# Autodesk Inventor assembly: z_assembly
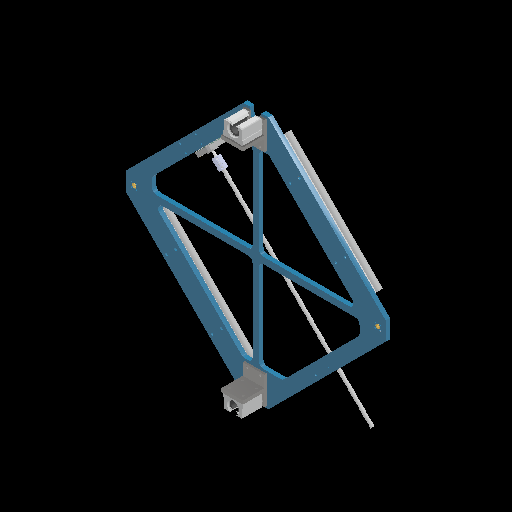
[picture p0: Inventor's stored thumbnail of the model, 512x512]
Saved by Autodesk Inventor 2026.1 (Build 301233000, 233)
## iProperties
Created: 2025-09-21
Part Number: z_assembly
Document SubType Name: Assembly
Designer: drago
Author: drago
## Documents named in this file (12)
- C:\Users\drago\Desktop\_QIST4500_Multidisciplinary_Team_Project\Proteox MX magnet positioner CAD\z_assembly\z_assembly.iam
- C:\Users\drago\Desktop\_QIST4500_Multidisciplinary_Team_Project\Proteox MX magnet positioner CAD\z_assembly\z_plate.ipt
- C:\Users\drago\Desktop\_QIST4500_Multidisciplinary_Team_Project\Proteox MX magnet positioner CAD\z_assembly\x_bearing_bracket.ipt
- C:\Users\drago\Desktop\_QIST4500_Multidisciplinary_Team_Project\Proteox MX magnet positioner CAD\z_assembly\z_bracket.ipt
- C:\Users\drago\Desktop\_QIST4500_Multidisciplinary_Team_Project\Proteox MX magnet positioner CAD\z_assembly\x_rail.ipt
- C:\Users\drago\Desktop\_QIST4500_Multidisciplinary_Team_Project\Proteox MX magnet positioner CAD\z_assembly\x_motor_bracket.ipt
- C:\Users\drago\Desktop\_QIST4500_Multidisciplinary_Team_Project\Proteox MX magnet positioner CAD\other_parts\KP08.iam
- C:\Users\drago\Desktop\_QIST4500_Multidisciplinary_Team_Project\Proteox MX magnet positioner CAD\other_parts\SBR16UU.ipt
- C:\Users\drago\Desktop\_QIST4500_Multidisciplinary_Team_Project\Proteox MX magnet positioner CAD\other_parts\Trapezoidal lead screw Nut tr8x8-4.ipt
- C:\Users\drago\Desktop\_QIST4500_Multidisciplinary_Team_Project\Proteox MX magnet positioner CAD\other_parts\Stepping_Motor_Nema17_34mm.ipt
- C:\Users\drago\Desktop\_QIST4500_Multidisciplinary_Team_Project\Proteox MX magnet positioner CAD\other_parts\5X8_COUPLER.ipt
- C:\Users\drago\Desktop\_QIST4500_Multidisciplinary_Team_Project\Proteox MX magnet positioner CAD\other_parts\Lead Screw 8mm-2.0 x 500mm.ipt
## Components (15 placed, 11 different names)
1. z_plate:1 — Mate:41, Mate:42, Mate:65, Mate:69, Mate:70, Mate:71, Mate:72, Mate:73, Mate:74, Mate:75, Mate:76, Mate:77, Mate:78, Mate:79, Mate:80, Mate:81, Mate:95, Mate:96, Mate:97, Mate:98, Mate:99, Mate:100, Mate:107, Mate:108, Mate:109
2. x_bearing_bracket:1 — Mate:65, Mate:84, Mate:85, Mate:86, Mate:109
3. z_bracket:1 — Mate:75, Mate:77, Mate:78, Mate:87, Mate:89, Mate:90
4. x_rail:1 — Mate:72, Mate:73, Mate:74
5. z_bracket:2 — Mate:76, Mate:79, Mate:80, Mate:88, Mate:91, Mate:92
6. x_rail:2 — Mate:69, Mate:70, Mate:71
7. x_motor_bracket:1 — Mate:81, Mate:101, Mate:102, Mate:103, Mate:107, Mate:108
8. KP08:1 [sub-assembly] — Mate:84, Mate:85, Mate:86, Mate:105
9. SBR16UU:1 — Mate:87, Mate:89, Mate:90
10. SBR16UU:2 — Mate:88, Mate:91, Mate:92
11. Trapezoidal lead screw Nut tr8x8-4:1 — Mate:95, Mate:96, Mate:97
12. Trapezoidal lead screw Nut tr8x8-4:2 — Mate:98, Mate:99, Mate:100
13. Stepping_Motor_Nema17_34mm:1 — Mate:93, Mate:94, Mate:101, Mate:102, Mate:103, Mate:106
14. 5X8_COUPLER:1 — Mate:93, Mate:94, Mate:104
15. Lead Screw 8mm-2.0 x 500mm:1 — Mate:104, Mate:105, Mate:106
## Relationships (42: Mate 42)
- Mate:41: z_plate:1
- Mate:42: z_plate:1
- Mate:65: z_plate:1 ↔ x_bearing_bracket:1
- Mate:69: z_plate:1 ↔ x_rail:2
- Mate:70: z_plate:1 ↔ x_rail:2
- Mate:71: z_plate:1 ↔ x_rail:2
- Mate:72: z_plate:1 ↔ x_rail:1
- Mate:73: z_plate:1 ↔ x_rail:1
- Mate:74: z_plate:1 ↔ x_rail:1
- Mate:75: z_plate:1 ↔ z_bracket:1
- Mate:76: z_plate:1 ↔ z_bracket:2
- Mate:77: z_plate:1 ↔ z_bracket:1
- Mate:78: z_plate:1 ↔ z_bracket:1
- Mate:79: z_plate:1 ↔ z_bracket:2
- Mate:80: z_plate:1 ↔ z_bracket:2
- Mate:81: z_plate:1 ↔ x_motor_bracket:1
- Mate:84: x_bearing_bracket:1 ↔ KP08:1
- Mate:85: x_bearing_bracket:1 ↔ KP08:1
- Mate:86: x_bearing_bracket:1 ↔ KP08:1
- Mate:87: z_bracket:1 ↔ SBR16UU:1
- Mate:88: z_bracket:2 ↔ SBR16UU:2
- Mate:89: z_bracket:1 ↔ SBR16UU:1
- Mate:90: z_bracket:1 ↔ SBR16UU:1
- Mate:91: z_bracket:2 ↔ SBR16UU:2
- Mate:92: z_bracket:2 ↔ SBR16UU:2
- Mate:93: Stepping_Motor_Nema17_34mm:1 ↔ 5X8_COUPLER:1
- Mate:94 (10 mm): Stepping_Motor_Nema17_34mm:1 ↔ 5X8_COUPLER:1
- Mate:95: z_plate:1 ↔ Trapezoidal lead screw Nut tr8x8-4:1
- Mate:96: z_plate:1 ↔ Trapezoidal lead screw Nut tr8x8-4:1
- Mate:97: z_plate:1 ↔ Trapezoidal lead screw Nut tr8x8-4:1
- Mate:98: z_plate:1 ↔ Trapezoidal lead screw Nut tr8x8-4:2
- Mate:99: z_plate:1 ↔ Trapezoidal lead screw Nut tr8x8-4:2
- Mate:100: z_plate:1 ↔ Trapezoidal lead screw Nut tr8x8-4:2
- Mate:101: x_motor_bracket:1 ↔ Stepping_Motor_Nema17_34mm:1
- Mate:102: x_motor_bracket:1 ↔ Stepping_Motor_Nema17_34mm:1
- Mate:103: x_motor_bracket:1 ↔ Stepping_Motor_Nema17_34mm:1
- Mate:104: 5X8_COUPLER:1 ↔ Lead Screw 8mm-2.0 x 500mm:1
- Mate:105: KP08:1 ↔ Lead Screw 8mm-2.0 x 500mm:1
- Mate:106: Stepping_Motor_Nema17_34mm:1 ↔ Lead Screw 8mm-2.0 x 500mm:1
- Mate:107: z_plate:1 ↔ x_motor_bracket:1
- Mate:108: z_plate:1 ↔ x_motor_bracket:1
- Mate:109: z_plate:1 ↔ x_bearing_bracket:1
